# Autodesk Inventor assembly: Tapeta exterior con tornillos
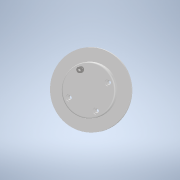
[picture p0: Inventor's stored thumbnail of the model, 180x180]
Saved by Autodesk Inventor 2021 (Build 250183000, 183)
## iProperties
Created: 2021-01-10
Part Number: Tapeta exterior con tornillos
Document SubType Name: Assembly
Designer: dieku
Author: dieku
## Documents named in this file (3)
- C:\Users\dieku\Documents\GitHub\tallerDibujoIngenieria\Ensambles\Tapeta exterior con tornillos.iam
- C:\Users\dieku\Documents\GitHub\tallerDibujoIngenieria\Partes\Tapeta Exterior.ipt
- C:\Users\dieku\Documents\Inventor\Content Center Files\R2021\en-US\DIN 912\DIN 912 - M6 x 1 x 25 x 22,5.ipt
## Components (2 placed, 2 different names)
1. Tapeta Exterior:1 — Insert:1
2. DIN 912 - replaced by DIN EN ISO 4762 M6 x 25:1 — Insert:1
## Relationships (1: Insert 1)
- Insert:1: Tapeta Exterior:1 ↔ DIN 912 - replaced by DIN EN ISO 4762 M6 x 25:1
